# Autodesk Inventor assembly: 2017 Chassis
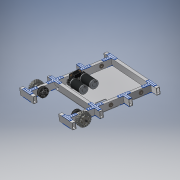
[picture p0: Inventor's stored thumbnail of the model, 180x180]
Saved by Autodesk Inventor 2016 (Build 200138000, 138)
## iProperties
Created: 2017-01-08
Part Number: 2017 Chassis
Document SubType Name: Assembly
Designer: Dhruv
Author: Dhruv
## Documents named in this file (7)
- C:\Users\Dhruv\Desktop\MISC\FRC 2017\2017 Chassis.iam
- C:\Users\Dhruv\Desktop\MISC\FRC 2017\Chassie2.iam
- C:\Users\Dhruv\Desktop\MISC\FRC 2017\supporting_parts\217-3875-STEP-20140818.ipt
- C:\Users\Dhruv\Desktop\MISC\FRC 2017\supporting_parts\FrontWheelAssembly.iam
- C:\Users\Dhruv\Desktop\MISC\FRC 2017\supporting_parts\CIMWithGearBox.iam
- C:\Users\Dhruv\Desktop\MISC\FRC 2017\supporting_parts\217-3550-STEP.ipt
- C:\Users\Dhruv\Desktop\MISC\FRC 2017\supporting_parts\217-3547-STEP.ipt
## Components (28 placed, 6 different names)
1. Chassie2:1 [sub-assembly] — Insert:3, Insert:4, Insert:5, Insert:6, Insert:7, Insert:8, Insert:9, Insert:10, Insert:11, Mate:2, Flush:1, Flush:2, Mate:3, Flush:3, Flush:4, Mate:4, Flush:5, Flush:6, Mate:5, Flush:7, Flush:8, Mate:6, Flush:9, Flush:10, Mate:7, Flush:11, Flush:12, Mate:8, Flush:13, Flush:14, Mate:9, Flush:15, Flush:16, Mate:10, Flush:17, Flush:18, Mate:11, Flush:19, Flush:20, Mate:12, Flush:21, Flush:22, Mate:13, Flush:23, Flush:24, Mate:14, Flush:25, Flush:26, Mate:15, Flush:27, Flush:28, Mate:16, Flush:29, Flush:30, Mate:17, Flush:31, Flush:32
2. 217-3875-STEP-20140818:3 — Insert:3
3. 217-3875-STEP-20140818:4 — Insert:4
4. 217-3875-STEP-20140818:5 — Insert:5
5. 217-3875-STEP-20140818:6 — Insert:6
6. 217-3875-STEP-20140818:7 — Insert:8
7. 217-3875-STEP-20140818:8 — Insert:7
8. 217-3875-STEP-20140818:9 — Insert:9
9. 217-3875-STEP-20140818:10 — Insert:10, Mate:1
10. FrontWheelAssembly:1 [sub-assembly]
11. FrontWheelAssembly:2 [sub-assembly] — Insert:11
12. CIMWithGearBox:1 [sub-assembly] — Mate:1
13. 217-3550-STEP:1 — Mate:4, Flush:5, Flush:6
14. 217-3547-STEP:1 — Mate:2, Flush:1, Flush:2
15. 217-3547-STEP:2 — Mate:3, Flush:3, Flush:4
16. 217-3550-STEP:2 — Mate:5, Flush:7, Flush:8
17. 217-3547-STEP:3 — Mate:8, Flush:13, Flush:14
18. 217-3547-STEP:4 — Mate:9, Flush:15, Flush:16
19. 217-3547-STEP:5 — Mate:6, Flush:9, Flush:10
20. 217-3547-STEP:6 — Mate:7, Flush:11, Flush:12
21. 217-3547-STEP:7 — Mate:10, Flush:17, Flush:18
22. 217-3547-STEP:8 — Mate:11, Flush:19, Flush:20
23. 217-3547-STEP:9 — Mate:12, Flush:21, Flush:22
24. 217-3547-STEP:10 — Mate:13, Flush:23, Flush:24
25. 217-3547-STEP:11 — Mate:15, Flush:27, Flush:28
26. 217-3547-STEP:12 — Mate:14, Flush:25, Flush:26
27. 217-3547-STEP:13 — Mate:16, Flush:29, Flush:30
28. 217-3547-STEP:14 — Mate:17, Flush:31, Flush:32
## Relationships (60: Flush 32, Mate 17, Insert 11)
- [Insert]: Chassie2:1 ↔ FrontWheelAssembly:1
- [Insert]: Chassie2:1 ↔ FrontWheelAssembly:1
- Insert:3: Chassie2:1 ↔ 217-3875-STEP-20140818:3
- Insert:4: Chassie2:1 ↔ 217-3875-STEP-20140818:4
- Insert:5: Chassie2:1 ↔ 217-3875-STEP-20140818:5
- Insert:6: Chassie2:1 ↔ 217-3875-STEP-20140818:6
- Insert:7: Chassie2:1 ↔ 217-3875-STEP-20140818:8
- Insert:8: Chassie2:1 ↔ 217-3875-STEP-20140818:7
- Insert:9: Chassie2:1 ↔ 217-3875-STEP-20140818:9
- Insert:10: Chassie2:1 ↔ 217-3875-STEP-20140818:10
- Insert:11: Chassie2:1 ↔ FrontWheelAssembly:2
- Mate:1: 217-3875-STEP-20140818:10 ↔ CIMWithGearBox:1
- Mate:2: Chassie2:1 ↔ 217-3547-STEP:1
- Flush:1: Chassie2:1 ↔ 217-3547-STEP:1
- Flush:2: Chassie2:1 ↔ 217-3547-STEP:1
- Mate:3: Chassie2:1 ↔ 217-3547-STEP:2
- Flush:3: Chassie2:1 ↔ 217-3547-STEP:2
- Flush:4: Chassie2:1 ↔ 217-3547-STEP:2
- Mate:4: Chassie2:1 ↔ 217-3550-STEP:1
- Flush:5: Chassie2:1 ↔ 217-3550-STEP:1
- Flush:6: Chassie2:1 ↔ 217-3550-STEP:1
- Mate:5: Chassie2:1 ↔ 217-3550-STEP:2
- Flush:7: Chassie2:1 ↔ 217-3550-STEP:2
- Flush:8: Chassie2:1 ↔ 217-3550-STEP:2
- Mate:6: Chassie2:1 ↔ 217-3547-STEP:5
- Flush:9: Chassie2:1 ↔ 217-3547-STEP:5
- Flush:10: Chassie2:1 ↔ 217-3547-STEP:5
- Mate:7: Chassie2:1 ↔ 217-3547-STEP:6
- Flush:11: Chassie2:1 ↔ 217-3547-STEP:6
- Flush:12: Chassie2:1 ↔ 217-3547-STEP:6
- Mate:8: Chassie2:1 ↔ 217-3547-STEP:3
- Flush:13: Chassie2:1 ↔ 217-3547-STEP:3
- Flush:14: Chassie2:1 ↔ 217-3547-STEP:3
- Mate:9: Chassie2:1 ↔ 217-3547-STEP:4
- Flush:15: Chassie2:1 ↔ 217-3547-STEP:4
- Flush:16: Chassie2:1 ↔ 217-3547-STEP:4
- Mate:10: Chassie2:1 ↔ 217-3547-STEP:7
- Flush:17: Chassie2:1 ↔ 217-3547-STEP:7
- Flush:18: Chassie2:1 ↔ 217-3547-STEP:7
- Mate:11: Chassie2:1 ↔ 217-3547-STEP:8
- Flush:19: Chassie2:1 ↔ 217-3547-STEP:8
- Flush:20: Chassie2:1 ↔ 217-3547-STEP:8
- Mate:12: Chassie2:1 ↔ 217-3547-STEP:9
- Flush:21: Chassie2:1 ↔ 217-3547-STEP:9
- Flush:22: Chassie2:1 ↔ 217-3547-STEP:9
- Mate:13: Chassie2:1 ↔ 217-3547-STEP:10
- Flush:23: Chassie2:1 ↔ 217-3547-STEP:10
- Flush:24: Chassie2:1 ↔ 217-3547-STEP:10
- Mate:14: Chassie2:1 ↔ 217-3547-STEP:12
- Flush:25: Chassie2:1 ↔ 217-3547-STEP:12
- Flush:26: Chassie2:1 ↔ 217-3547-STEP:12
- Mate:15: Chassie2:1 ↔ 217-3547-STEP:11
- Flush:27: Chassie2:1 ↔ 217-3547-STEP:11
- Flush:28: Chassie2:1 ↔ 217-3547-STEP:11
- Mate:16: Chassie2:1 ↔ 217-3547-STEP:13
- Flush:29: Chassie2:1 ↔ 217-3547-STEP:13
- Flush:30: Chassie2:1 ↔ 217-3547-STEP:13
- Mate:17: Chassie2:1 ↔ 217-3547-STEP:14
- Flush:31: Chassie2:1 ↔ 217-3547-STEP:14
- Flush:32: Chassie2:1 ↔ 217-3547-STEP:14
